# Autodesk Inventor assembly: Pincher_SOLID
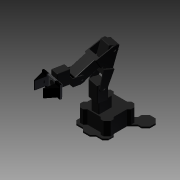
[picture p0: Inventor's stored thumbnail of the model, 180x180]
Saved by Autodesk Inventor 2012 (Build 160160000, 160)
## iProperties
Created: 2013-03-08
Part Number: Pincher_SOLID
Document SubType Name: Assembly
Designer: Andrew
Author: Andrew
## Documents named in this file (6)
- R:\PhantomX Pincher Arm\Pincher_SOLID\Pincher_SOLID.iam
- R:\PhantomX Pincher Arm\Pincher_SOLID\Base.ipt
- R:\PhantomX Pincher Arm\Pincher_SOLID\Shoulder.ipt
- R:\PhantomX Pincher Arm\Pincher_SOLID\Bicep.ipt
- R:\PhantomX Pincher Arm\Pincher_SOLID\PX-Gripper.iam
- R:\PhantomX Pincher Arm\Pincher_SOLID\Wrist.ipt
## Components (6 placed, 5 different names)
1. Base:1 — Insert:1, Angle:2
2. Shoulder:1 — Insert:1, Insert:2
3. Bicep:1 — Insert:2, Insert:3
4. Bicep:2 — Insert:3, Insert:4
5. PX-Gripper:1 [sub-assembly] — Insert:5, Angle:1
6. Wrist:1 — Insert:4, Insert:5, Angle:1, Angle:2
## Relationships (7: Insert 5, Angle 2)
- Insert:1: Base:1 ↔ Shoulder:1
- Insert:2: Shoulder:1 ↔ Bicep:1
- Insert:3: Bicep:1 ↔ Bicep:2
- Insert:4: Bicep:2 ↔ Wrist:1
- Insert:5: PX-Gripper:1 ↔ Wrist:1
- Angle:1 (0 deg): PX-Gripper:1 ↔ Wrist:1
- Angle:2 (0 deg): Base:1 ↔ Wrist:1
